# Autodesk Inventor assembly: BOX_CETIN
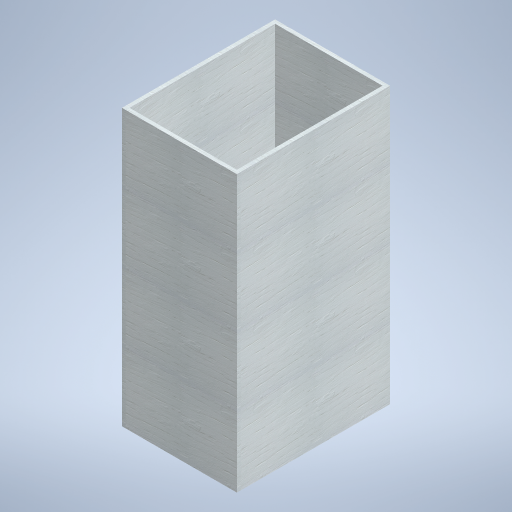
[picture p0: Inventor's stored thumbnail of the model, 512x512]
Saved by Autodesk Inventor 2023 (Build 270158000, 158)
## iProperties
Created: 2024-02-20
Part Number: BOX_CETIN
Document SubType Name: Assembly
Designer: vraco
Author: vraco
## Documents named in this file (4)
- C:\Users\vraco\Documents\Inventor\kos_e-cigarety\BOX_CETIN.iam
- C:\Users\vraco\Documents\Inventor\kos_e-cigarety\BOTTOM_CETIN_PART_BOX.ipt
- C:\Users\vraco\Documents\Inventor\kos_e-cigarety\FRONT_SIDE_CETIN_PART_BOX.ipt
- C:\Users\vraco\Documents\Inventor\kos_e-cigarety\SIDE_CETIN_PART_BOX.ipt
## Components (5 placed, 3 different names)
1. BOTTOM_CETIN_PART_BOX:1 — Flush:1, Flush:2, Flush:3, Mate:1, Mate:2, Mate:3, Mate:5, Mate:7
2. FRONT_SIDE_CETIN_PART_BOX:1 — Flush:4, Mate:1, Mate:2, Mate:4, Mate:6
3. SIDE_CETIN_PART_BOX:1 — Flush:5, Mate:3, Mate:4, Mate:8
4. SIDE_CETIN_PART_BOX:2 — Flush:6, Mate:5, Mate:6
5. FRONT_SIDE_CETIN_PART_BOX:2 — Flush:7, Mate:7, Mate:8
## Relationships (15: Mate 8, Flush 7)
- Flush:1: BOTTOM_CETIN_PART_BOX:1
- Flush:2: BOTTOM_CETIN_PART_BOX:1
- Flush:3: BOTTOM_CETIN_PART_BOX:1
- Flush:4: FRONT_SIDE_CETIN_PART_BOX:1
- Mate:1: BOTTOM_CETIN_PART_BOX:1 ↔ FRONT_SIDE_CETIN_PART_BOX:1
- Mate:2: BOTTOM_CETIN_PART_BOX:1 ↔ FRONT_SIDE_CETIN_PART_BOX:1
- Flush:5: SIDE_CETIN_PART_BOX:1
- Mate:3: BOTTOM_CETIN_PART_BOX:1 ↔ SIDE_CETIN_PART_BOX:1
- Mate:4: FRONT_SIDE_CETIN_PART_BOX:1 ↔ SIDE_CETIN_PART_BOX:1
- Flush:6: SIDE_CETIN_PART_BOX:2
- Mate:5: BOTTOM_CETIN_PART_BOX:1 ↔ SIDE_CETIN_PART_BOX:2
- Mate:6: FRONT_SIDE_CETIN_PART_BOX:1 ↔ SIDE_CETIN_PART_BOX:2
- Flush:7: FRONT_SIDE_CETIN_PART_BOX:2
- Mate:7: BOTTOM_CETIN_PART_BOX:1 ↔ FRONT_SIDE_CETIN_PART_BOX:2
- Mate:8: SIDE_CETIN_PART_BOX:1 ↔ FRONT_SIDE_CETIN_PART_BOX:2
